# Autodesk Inventor assembly: 2 in 30A flex wheel LS mount
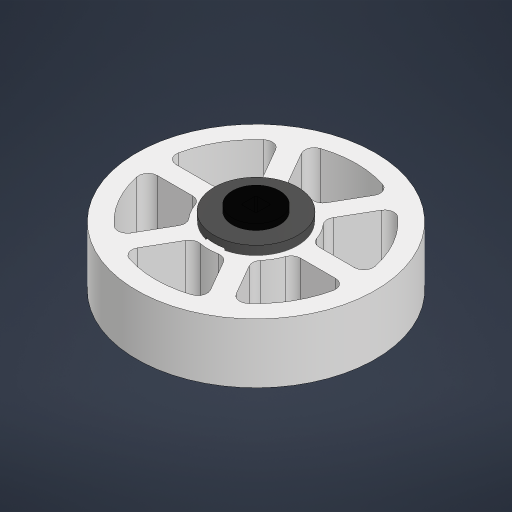
[picture p0: Inventor's stored thumbnail of the model, 512x512]
Saved by Autodesk Inventor 2023.2 (Build 272271030, 271C)
## iProperties
Created: 2023-03-24
Part Number: 2 in 30A flex wheel LS mount
Document SubType Name: Assembly
Designer: Main Account
Author: Main Account
## Documents named in this file (5)
- C:\Users\Main Account\InventorProjects\VEX\Custom Library\2 in 30A flex wheel LS mount.iam
- C:\Users\Main Account\InventorProjects\VEX\Library Backup\Library 1.4\Motion\Wheels\Flex Wheels\2.000 Flex Wheel.ipt
- C:\Users\Main Account\InventorProjects\VEX\Library Backup\Library 1.4\Motion\Wheels\Flex Wheels\VersaHex Adapters .250.ipt
- C:\Users\Main Account\InventorProjects\VEX\Library Backup\Library 1.4\Motion\Insert Square.ipt
- C:\Users\Main Account\InventorProjects\VEX\Library Backup\Library 1.4\Motion\Wheels\Flex Wheels\2.000 Flex Wheel\2.000 30A .500.ipt
## Components (5 placed, 3 different names)
1. 2.000 30A .500:1 — Mate:5, Mate:6, Mate:7, Mate:8, Angle:2
2. VersaHex Adapters .250:1 — Mate:1, Mate:2, Mate:5, Mate:6, Angle:1
3. VersaHex Adapters .250:2 — Mate:3, Mate:4, Mate:7, Mate:8, Angle:1, Angle:2
4. Insert Square:1 — Mate:1, Mate:2
5. Insert Square:2 — Mate:3, Mate:4
## Relationships (10: Mate 8, Angle 2)
- Mate:1: VersaHex Adapters .250:1 ↔ Insert Square:1
- Mate:2: VersaHex Adapters .250:1 ↔ Insert Square:1
- Mate:3: VersaHex Adapters .250:2 ↔ Insert Square:2
- Mate:4: VersaHex Adapters .250:2 ↔ Insert Square:2
- Mate:5 (-0.465 mm): 2.000 30A .500:1 ↔ VersaHex Adapters .250:1
- Mate:6: 2.000 30A .500:1 ↔ VersaHex Adapters .250:1
- Mate:7 (-0.465 mm): 2.000 30A .500:1 ↔ VersaHex Adapters .250:2
- Mate:8: 2.000 30A .500:1 ↔ VersaHex Adapters .250:2
- Angle:1 (0 deg): VersaHex Adapters .250:1 ↔ VersaHex Adapters .250:2
- Angle:2 (0 deg): 2.000 30A .500:1 ↔ VersaHex Adapters .250:2
